# Autodesk Inventor assembly: intake with drivebase
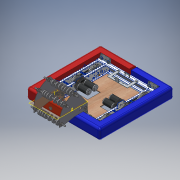
[picture p0: Inventor's stored thumbnail of the model, 180x180]
Saved by Autodesk Inventor 2018 (Build 220112000, 112)
## iProperties
Created: 2020-01-24
Part Number: intake with drivebase
Document SubType Name: Assembly
Designer: s-2513225
Author: s-2513225
## Documents named in this file (3)
- \\studenthome\students\S-2513225\GitHub\2020CAD\Over bumper intake\Assembly\intake with drivebase.iam
- \\studenthome\students\S-2513225\GitHub\2020CAD\Over bumper intake\Assembly\waterjet assembly version.iam
- \\studenthome\students\S-2513225\GitHub\2020CAD\Drivebase AM14U1\Main Assembly File\Drivebase AM14U4 Square 28inx28in.iam
## Components (3 placed, 2 different names)
1. waterjet assembly version:1 [sub-assembly] — Mate:1, Mate:2, Flush:1, Mate:5
2. Drivebase AM14U4 Square 28inx28in:1 [sub-assembly] — Mate:1, Mate:2, Flush:1, Mate:4
3. waterjet assembly version:2 [sub-assembly] — Mate:4, Mate:5
## Relationships (5: Mate 4, Flush 1)
- Mate:1: waterjet assembly version:1 ↔ Drivebase AM14U4 Square 28inx28in:1
- Mate:2 (203.2 mm): waterjet assembly version:1 ↔ Drivebase AM14U4 Square 28inx28in:1
- Flush:1: waterjet assembly version:1 ↔ Drivebase AM14U4 Square 28inx28in:1
- Mate:4 (203.2 mm): Drivebase AM14U4 Square 28inx28in:1 ↔ waterjet assembly version:2
- Mate:5: waterjet assembly version:1 ↔ waterjet assembly version:2
